# Autodesk Inventor assembly: Robot Assembly
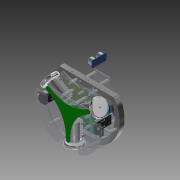
[picture p0: Inventor's stored thumbnail of the model, 180x180]
Saved by Autodesk Inventor 2015 (Build 190159000, 159)
## iProperties
Created: 2016-02-17
Part Number: Robot Assembly
Document SubType Name: Assembly
Designer: 23902
Author: 23902
## Documents named in this file (29)
- C:\Users\23902\git\Work\Design\3D Printing\Version 4\Robot Assembly.iam
- C:\Users\23902\git\Work\Design\3D Printing\Version 4\Motor Mount Plate.ipt
- C:\Users\23902\git\Work\Design\3D Printing\Motor Mount Bracket.ipt
- C:\Users\23902\git\Work\Design\3D Printing\Motor.ipt
- C:\Users\23902\git\Work\Design\3D Printing\Wheel.ipt
- C:\Users\23902\git\Work\Design\3D Printing\Version 4\Middle Plate.ipt
- C:\Users\23902\git\Work\Design\3D Printing\Ball.ipt
- C:\Users\23902\git\Work\Design\3D Printing\Version 4\Standoff 20.ipt
- C:\Users\23902\git\Work\Design\3D Printing\Version 4\Light Sensor Plate.ipt
- C:\Users\23902\git\Work\Design\3D Printing\Version 4\Light Sensor PCB.ipt
- C:\Users\23902\git\Work\Design\3D Printing\Version 4\Standoff 10.ipt
- C:\Users\23902\git\Work\Design\3D Printing\ArduinoMEGA2560.ipt
- C:\Users\23902\git\Work\Design\3D Printing\Version 4\Standoff 30.ipt
- C:\Users\23902\git\Work\Design\3D Printing\Version 4\Veroboard.ipt
- C:\Users\23902\git\Work\Design\3D Printing\Version 4\M3x20 Screw Nylon.ipt
- C:\Users\23902\git\Work\Design\3D Printing\Version 4\M3x10 Screw Nylon.ipt
- C:\Users\23902\git\Work\Design\3D Printing\Version 4\M3x6 Screw Nylon.ipt
- C:\Users\23902\git\Work\Design\3D Printing\Version 4\M3 Nut Nylon.ipt
- C:\Users\23902\git\Work\Design\3D Printing\Version 4\M3x10 Screw Steel.ipt
- C:\Users\23902\git\Work\Design\3D Printing\Version 4\M3 Nut Steel.ipt
- C:\Users\23902\git\Work\Design\3D Printing\Version 4\Battery.ipt
- C:\Users\23902\git\Work\Design\3D Printing\Version 4\Top Plate.ipt
- C:\Users\23902\git\Work\Design\3D Printing\Digit Display.ipt
- C:\Users\23902\git\Work\Design\3D Printing\HC-SR04 Sonar.ipt
- C:\Users\23902\git\Work\Design\3D Printing\Version 4\Sonar Mount.ipt
- C:\Users\23902\git\Work\Design\3D Printing\Version 4\Standoff 40.ipt
- C:\Users\23902\git\Work\Design\3D Printing\Compass.ipt
- C:\Users\23902\git\Work\Design\3D Printing\Version 4\M2x10 Screw Steel.ipt
- C:\Users\23902\git\Work\Design\3D Printing\Version 4\M2 Nut Steel.ipt
## Components (131 placed, 28 different names)
1. Motor Mount Plate:1 — Mate:1, Mate:2, Mate:3, Mate:22, Mate:23, Mate:24, Mate:25, Mate:26, Mate:27, Mate:28, Mate:29, Mate:30, Mate:31, Mate:32, Mate:33, Mate:34, Mate:35, Mate:101, Mate:102, Mate:103, Mate:104, Mate:113, Mate:114, Mate:115, Mate:116, Mate:117, Mate:118, Mate:127, Mate:128, Mate:129, Mate:130, Mate:131, Mate:132, Mate:155, Mate:156, Mate:157, Mate:158, Mate:159, Mate:160, Mate:161, Mate:162, Mate:182, Mate:183, Mate:184, Mate:185, Mate:186, Mate:187, Mate:203, Mate:204, Mate:205, Mate:206, Mate:207, Mate:208, Mate:209, Mate:210, Mate:211, Mate:212, Mate:213, Mate:214, Mate:223, Mate:224, Mate:225, Mate:226, Mate:227, Mate:228, Mate:229, Mate:230, Mate:249, Mate:250, Mate:251, Mate:252, Mate:253, Mate:254, Mate:255, Mate:256, Mate:257, Mate:269, Mate:270, Mate:272, Mate:274, Mate:278, Mate:280, Mate:281, Mate:282, Mate:284, Mate:288, Mate:289, Mate:290, Mate:291, Mate:293, Mate:294, Mate:295, Mate:296, Mate:297, Mate:298, Mate:299, Mate:300, Mate:301, Mate:302, Mate:303
2. Motor Mount Bracket:1 — Mate:1, Mate:11, Mate:14, Mate:15, Mate:24, Mate:25, Mate:275, Mate:276, Mate:286, Mate:287
3. Motor:1 — Mate:10, Mate:16, Mate:17, Mate:21, Flush:3
4. Wheel:1 — Mate:19, Flush:1
5. Motor Mount Bracket:2 — Mate:2, Mate:10, Mate:16, Mate:17, Mate:22, Mate:23, Mate:267, Mate:268, Mate:277, Mate:279
6. Motor:2 — Mate:11, Mate:14, Mate:15, Mate:19, Flush:1
7. Wheel:2 — Mate:20, Flush:2
8. Motor Mount Bracket:3 — Mate:3, Mate:12, Mate:13, Mate:18, Mate:26, Mate:27, Mate:271, Mate:273, Mate:283, Mate:285
9. Motor:3 — Mate:12, Mate:13, Mate:18, Mate:20, Flush:2
10. Wheel:3 — Mate:21, Flush:3
11. Middle Plate:1 — Mate:36, Mate:37, Mate:38, Mate:191, Mate:192, Mate:193, Mate:194, Mate:195, Mate:196, Mate:197, Mate:198, Mate:199, Mate:200, Mate:201, Mate:202, Mate:315, Mate:316, Mate:317, Mate:318, Mate:319, Mate:320, Mate:321, Mate:322, Mate:323, Mate:324, Mate:325, Mate:326, Mate:327, Mate:328, Mate:329, Mate:330
12. Ball:1
13. Standoff 20:1 — Mate:28, Mate:33, Mate:38
14. Standoff 20:2 — Mate:29, Mate:35, Mate:36
15. Standoff 20:3 — Mate:31, Mate:32
16. Standoff 20:4 — Mate:30, Mate:34, Mate:37
17. Light Sensor Plate:1 — Mate:152, Mate:153, Mate:154, Mate:163, Mate:164, Mate:165, Mate:215, Mate:216, Mate:217, Mate:218, Mate:219, Mate:220, Mate:221, Mate:222, Mate:362, Mate:384, Mate:385, Mate:386, Mate:387, Mate:388, Mate:389, Mate:390, Mate:391, Mate:392, Mate:393, Mate:394, Mate:395, Mate:396
18. Light Sensor PCB:1 — Mate:152, Mate:153, Mate:154
19. Standoff 20:5 — Mate:103, Mate:104
20. Standoff 20:6 — Mate:101, Mate:102
21. Standoff 10:1 — Mate:114, Mate:128, Mate:263
22. Standoff 10:2 — Mate:115, Mate:129, Mate:266
23. Standoff 10:3 — Mate:116, Mate:130, Mate:133, Mate:260
24. Standoff 10:4 — Mate:118, Mate:131, Mate:259
25. Standoff 10:5 — Mate:117, Mate:126, Mate:132, Mate:261
26. Standoff 10:6 — Mate:113, Mate:125, Mate:127, Mate:265
27. -  -:1 — Mate:125, Mate:126, Mate:133, Mate:234, Mate:235, Mate:236, Mate:237, Mate:238, Mate:239, Mate:240, Mate:241, Mate:242, Mate:243, Mate:244, Mate:245
28. Standoff 30:1 — Mate:157, Mate:162
29. Standoff 30:2 — Mate:159, Mate:161
30. Standoff 30:3 — Mate:155, Mate:156, Mate:163, Mate:164
31. Standoff 30:4 — Mate:158, Mate:160, Mate:165
32. Standoff 10:7 — Mate:182, Mate:186, Mate:190, Mate:258
33. Standoff 10:8 — Mate:183, Mate:187, Mate:188, Mate:189, Mate:262
34. Standoff 10:9 — Mate:184, Mate:185, Mate:264
35. Veroboard:1 — Mate:188, Mate:189, Mate:190, Mate:231, Mate:232, Mate:233, Mate:246, Mate:247, Mate:248
36. M3x20 Screw Nylon:1 — Mate:192, Mate:201
37. M3x20 Screw Nylon:2 — Mate:193, Mate:202
38. M3x20 Screw Nylon:3 — Mate:194, Mate:199
39. M3x20 Screw Nylon:4 — Mate:195, Mate:198
40. M3x20 Screw Nylon:5 — Mate:196, Mate:197
41. M3x20 Screw Nylon:6 — Mate:191, Mate:200
42. M3x10 Screw Nylon:1 — Mate:208, Mate:209
43. M3x10 Screw Nylon:2 — Mate:207, Mate:210
44. M3x10 Screw Nylon:3 — Mate:206, Mate:211
45. M3x10 Screw Nylon:4 — Mate:205, Mate:212
46. M3x10 Screw Nylon:5 — Mate:204, Mate:213
47. M3x10 Screw Nylon:6 — Mate:203, Mate:214
48. M3x10 Screw Nylon:7 — Mate:215, Mate:219
49. M3x10 Screw Nylon:8 — Mate:216, Mate:220
50. M3x10 Screw Nylon:9 — Mate:224, Mate:225
51. M3x10 Screw Nylon:10 — Mate:218, Mate:222
52. M3x10 Screw Nylon:11 — Mate:217, Mate:221
53. M3x10 Screw Nylon:12 — Mate:228, Mate:229
54. M3x10 Screw Nylon:13 — Mate:227, Mate:230
55. M3x10 Screw Nylon:14 — Mate:223, Mate:226
56. M3x6 Screw Nylon:1 — Mate:231, Mate:246
57. M3x6 Screw Nylon:2 — Mate:235, Mate:240
58. M3x6 Screw Nylon:3 — Mate:236, Mate:242
59. M3x6 Screw Nylon:4 — Mate:237, Mate:245
60. M3x6 Screw Nylon:5 — Mate:239, Mate:244
61. M3x6 Screw Nylon:6 — Mate:238, Mate:241
62. M3x6 Screw Nylon:7 — Mate:232, Mate:247
63. M3x6 Screw Nylon:8 — Mate:234, Mate:243
64. M3x6 Screw Nylon:9 — Mate:233, Mate:248
65. M3 Nut Nylon:1 — Mate:253, Mate:260
66. M3 Nut Nylon:2 — Mate:252, Mate:258
67. M3 Nut Nylon:3 — Mate:254, Mate:262
68. M3 Nut Nylon:4 — Mate:255, Mate:261
69. M3 Nut Nylon:5 — Mate:257, Mate:266
70. M3 Nut Nylon:6 — Mate:256, Mate:264
71. M3 Nut Nylon:7 — Mate:251, Mate:259
72. M3 Nut Nylon:8 — Mate:250, Mate:265
73. M3 Nut Nylon:9 — Mate:249, Mate:263
74. M3x10 Screw Steel:1 — Mate:271, Mate:272, Mate:292
75. M3x10 Screw Steel:2 — Mate:273, Mate:274, Mate:310
76. M3x10 Screw Steel:3 — Mate:268, Mate:269, Mate:307
77. M3x10 Screw Steel:4 — Mate:267, Mate:270, Mate:306
78. M3x10 Screw Steel:5 — Mate:283, Mate:284, Mate:308
79. M3x10 Screw Steel:6 — Mate:279, Mate:280, Mate:304
80. M3x10 Screw Steel:7 — Mate:277, Mate:278, Mate:305
81. M3x10 Screw Steel:8 — Mate:275, Mate:282, Mate:311
82. M3x10 Screw Steel:9 — Mate:287, Mate:288, Mate:314
83. M3x10 Screw Steel:10 — Mate:286, Mate:289, Mate:312
84. M3x10 Screw Steel:11 — Mate:285, Mate:290, Mate:309
85. M3x10 Screw Steel:12 — Mate:276, Mate:281, Mate:313
86. M3 Nut Steel:1 — Mate:295, Mate:314
87. M3 Nut Steel:2 — Mate:291, Mate:292
88. M3 Nut Steel:3 — Mate:294, Mate:312
89. M3 Nut Steel:4 — Mate:296, Mate:311
90. M3 Nut Steel:5 — Mate:298, Mate:310
91. M3 Nut Steel:6 — Mate:297, Mate:304
92. M3 Nut Steel:7 — Mate:300, Mate:305
93. M3 Nut Steel:8 — Mate:299, Mate:308
94. M3 Nut Steel:9 — Mate:301, Mate:306
95. M3 Nut Steel:10 — Mate:302, Mate:309
96. M3 Nut Steel:11 — Mate:293, Mate:313
97. M3 Nut Steel:12 — Mate:303, Mate:307
98. Battery:1
99. Standoff 30:5 — Mate:315, Mate:321
100. Standoff 30:6 — Mate:316, Mate:322, Mate:332
101. Standoff 30:7 — Mate:317, Mate:320, Mate:331, Mate:333
102. Standoff 30:8 — Mate:318, Mate:319
103. M3x20 Screw Nylon:7 — Mate:323, Mate:330
104. M3x20 Screw Nylon:8 — Mate:326, Mate:328
105. M3x20 Screw Nylon:9 — Mate:325, Mate:327
106. M3x20 Screw Nylon:10 — Mate:324, Mate:329
107. Top Plate:1 — Mate:331, Mate:332, Mate:333, Mate:334, Mate:335, Mate:336, Mate:337, Mate:338, Mate:339, Mate:340, Mate:341, Mate:342, Mate:343, Mate:344, Mate:356, Mate:357, Mate:358, Mate:359, Mate:365, Mate:366
108. M3x10 Screw Nylon:15 — Mate:335, Mate:339
109. M3x10 Screw Nylon:16 — Mate:334, Mate:340
110. M3x10 Screw Nylon:17 — Mate:337, Mate:341
111. M3x10 Screw Nylon:18 — Mate:336, Mate:338
112. Digit Display:1 — Mate:342, Mate:343, Mate:344
113. M3x10 Screw Nylon:19 — Mate:357, Mate:359, Mate:368
114. M3x10 Screw Nylon:21 — Mate:356, Mate:358, Mate:367
115. HC-SR04 Sonar:1 — Mate:360, Mate:361, Mate:376, Mate:377, Mate:380, Mate:381
116. Sonar Mount:1 — Mate:360, Mate:361, Mate:362, Mate:384, Mate:385
117. Standoff 40:3 — Mate:366, Mate:367, Mate:371
118. Standoff 40:4 — Mate:365, Mate:368, Mate:369, Mate:370
119. M3x10 Screw Nylon:22 — Mate:373, Mate:374
120. M3x10 Screw Nylon:23 — Mate:372, Mate:375
121. Compass:1 — Mate:369, Mate:370, Mate:371, Mate:372, Mate:373, Mate:374, Mate:375
122. M2x10 Screw Steel:1 — Mate:376, Mate:377, Mate:379
123. M2 Nut Steel:1 — Mate:379
124. M2 Nut Steel:2 — Mate:383
125. M2x10 Screw Steel:2 — Mate:380, Mate:381, Mate:383
126. HC-SR04 Sonar:2
127. Sonar Mount:2 — Mate:386, Mate:387, Mate:388
128. M3x10 Screw Nylon:24 — Mate:394, Mate:396
129. M3x10 Screw Nylon:25 — Mate:393, Mate:395
130. M3x10 Screw Nylon:26 — Mate:389, Mate:390
131. M3x10 Screw Nylon:27 — Mate:391, Mate:392
## Relationships (268: Mate 265, Flush 3)
- Mate:1: Motor Mount Plate:1 ↔ Motor Mount Bracket:1
- Mate:2: Motor Mount Plate:1 ↔ Motor Mount Bracket:2
- Mate:3: Motor Mount Plate:1 ↔ Motor Mount Bracket:3
- Mate:10: Motor:1 ↔ Motor Mount Bracket:2
- Mate:11: Motor Mount Bracket:1 ↔ Motor:2
- Mate:12: Motor Mount Bracket:3 ↔ Motor:3
- Mate:13: Motor Mount Bracket:3 ↔ Motor:3
- Mate:14: Motor Mount Bracket:1 ↔ Motor:2
- Mate:15: Motor Mount Bracket:1 ↔ Motor:2
- Mate:16: Motor:1 ↔ Motor Mount Bracket:2
- Mate:17: Motor:1 ↔ Motor Mount Bracket:2
- Mate:18: Motor Mount Bracket:3 ↔ Motor:3
- Mate:19: Wheel:1 ↔ Motor:2
- Flush:1: Wheel:1 ↔ Motor:2
- Mate:20: Wheel:2 ↔ Motor:3
- Flush:2: Wheel:2 ↔ Motor:3
- Mate:21: Motor:1 ↔ Wheel:3
- Flush:3: Motor:1 ↔ Wheel:3
- Mate:22: Motor Mount Plate:1 ↔ Motor Mount Bracket:2
- Mate:23: Motor Mount Plate:1 ↔ Motor Mount Bracket:2
- Mate:24: Motor Mount Plate:1 ↔ Motor Mount Bracket:1
- Mate:25: Motor Mount Plate:1 ↔ Motor Mount Bracket:1
- Mate:26: Motor Mount Plate:1 ↔ Motor Mount Bracket:3
- Mate:27: Motor Mount Plate:1 ↔ Motor Mount Bracket:3
- Mate:28: Motor Mount Plate:1 ↔ Standoff 20:1
- Mate:29: Motor Mount Plate:1 ↔ Standoff 20:2
- Mate:30: Motor Mount Plate:1 ↔ Standoff 20:4
- Mate:31: Motor Mount Plate:1 ↔ Standoff 20:3
- Mate:32: Motor Mount Plate:1 ↔ Standoff 20:3
- Mate:33: Motor Mount Plate:1 ↔ Standoff 20:1
- Mate:34: Motor Mount Plate:1 ↔ Standoff 20:4
- Mate:35: Motor Mount Plate:1 ↔ Standoff 20:2
- Mate:36: Middle Plate:1 ↔ Standoff 20:2
- Mate:37: Middle Plate:1 ↔ Standoff 20:4
- Mate:38: Middle Plate:1 ↔ Standoff 20:1
- Mate:101: Motor Mount Plate:1 ↔ Standoff 20:6
- Mate:102: Motor Mount Plate:1 ↔ Standoff 20:6
- Mate:103: Motor Mount Plate:1 ↔ Standoff 20:5
- Mate:104: Motor Mount Plate:1 ↔ Standoff 20:5
- Mate:113: Motor Mount Plate:1 ↔ Standoff 10:6
- Mate:114: Motor Mount Plate:1 ↔ Standoff 10:1
- Mate:115: Motor Mount Plate:1 ↔ Standoff 10:2
- Mate:116: Motor Mount Plate:1 ↔ Standoff 10:3
- Mate:117: Motor Mount Plate:1 ↔ Standoff 10:5
- Mate:118: Motor Mount Plate:1 ↔ Standoff 10:4
- Mate:125: Standoff 10:6 ↔ -  -:1
- Mate:126: Standoff 10:5 ↔ -  -:1
- Mate:127: Motor Mount Plate:1 ↔ Standoff 10:6
- Mate:128: Motor Mount Plate:1 ↔ Standoff 10:1
- Mate:129: Motor Mount Plate:1 ↔ Standoff 10:2
- Mate:130: Motor Mount Plate:1 ↔ Standoff 10:3
- Mate:131: Motor Mount Plate:1 ↔ Standoff 10:4
- Mate:132: Motor Mount Plate:1 ↔ Standoff 10:5
- Mate:133: Standoff 10:3 ↔ -  -:1
- Mate:152: Light Sensor Plate:1 ↔ Light Sensor PCB:1
- Mate:153: Light Sensor Plate:1 ↔ Light Sensor PCB:1
- Mate:154: Light Sensor Plate:1 ↔ Light Sensor PCB:1
- Mate:155: Motor Mount Plate:1 ↔ Standoff 30:3
- Mate:156: Motor Mount Plate:1 ↔ Standoff 30:3
- Mate:157: Motor Mount Plate:1 ↔ Standoff 30:1
- Mate:158: Motor Mount Plate:1 ↔ Standoff 30:4
- Mate:159: Motor Mount Plate:1 ↔ Standoff 30:2
- Mate:160: Motor Mount Plate:1 ↔ Standoff 30:4
- Mate:161: Motor Mount Plate:1 ↔ Standoff 30:2
- Mate:162: Motor Mount Plate:1 ↔ Standoff 30:1
- Mate:163: Light Sensor Plate:1 ↔ Standoff 30:3
- Mate:164: Light Sensor Plate:1 ↔ Standoff 30:3
- Mate:165: Light Sensor Plate:1 ↔ Standoff 30:4
- Mate:182: Motor Mount Plate:1 ↔ Standoff 10:7
- Mate:183: Motor Mount Plate:1 ↔ Standoff 10:8
- Mate:184: Motor Mount Plate:1 ↔ Standoff 10:9
- Mate:185: Motor Mount Plate:1 ↔ Standoff 10:9
- Mate:186: Motor Mount Plate:1 ↔ Standoff 10:7
- Mate:187: Motor Mount Plate:1 ↔ Standoff 10:8
- Mate:188: Standoff 10:8 ↔ Veroboard:1
- Mate:189: Standoff 10:8 ↔ Veroboard:1
- Mate:190: Standoff 10:7 ↔ Veroboard:1
- Mate:191: Middle Plate:1 ↔ M3x20 Screw Nylon:6
- Mate:192: Middle Plate:1 ↔ M3x20 Screw Nylon:1
- Mate:193: Middle Plate:1 ↔ M3x20 Screw Nylon:2
- Mate:194: Middle Plate:1 ↔ M3x20 Screw Nylon:3
- Mate:195: Middle Plate:1 ↔ M3x20 Screw Nylon:4
- Mate:196: Middle Plate:1 ↔ M3x20 Screw Nylon:5
- Mate:197: Middle Plate:1 ↔ M3x20 Screw Nylon:5
- Mate:198: Middle Plate:1 ↔ M3x20 Screw Nylon:4
- Mate:199: Middle Plate:1 ↔ M3x20 Screw Nylon:3
- Mate:200: Middle Plate:1 ↔ M3x20 Screw Nylon:6
- Mate:201: Middle Plate:1 ↔ M3x20 Screw Nylon:1
- Mate:202: Middle Plate:1 ↔ M3x20 Screw Nylon:2
- Mate:203: Motor Mount Plate:1 ↔ M3x10 Screw Nylon:6
- Mate:204: Motor Mount Plate:1 ↔ M3x10 Screw Nylon:5
- Mate:205: Motor Mount Plate:1 ↔ M3x10 Screw Nylon:4
- Mate:206: Motor Mount Plate:1 ↔ M3x10 Screw Nylon:3
- Mate:207: Motor Mount Plate:1 ↔ M3x10 Screw Nylon:2
- Mate:208: Motor Mount Plate:1 ↔ M3x10 Screw Nylon:1
- Mate:209: Motor Mount Plate:1 ↔ M3x10 Screw Nylon:1
- Mate:210: Motor Mount Plate:1 ↔ M3x10 Screw Nylon:2
- Mate:211: Motor Mount Plate:1 ↔ M3x10 Screw Nylon:3
- Mate:212: Motor Mount Plate:1 ↔ M3x10 Screw Nylon:4
- Mate:213: Motor Mount Plate:1 ↔ M3x10 Screw Nylon:5
- Mate:214: Motor Mount Plate:1 ↔ M3x10 Screw Nylon:6
- Mate:215: Light Sensor Plate:1 ↔ M3x10 Screw Nylon:7
- Mate:216: Light Sensor Plate:1 ↔ M3x10 Screw Nylon:8
- Mate:217: Light Sensor Plate:1 ↔ M3x10 Screw Nylon:11
- Mate:218: Light Sensor Plate:1 ↔ M3x10 Screw Nylon:10
- Mate:219: Light Sensor Plate:1 ↔ M3x10 Screw Nylon:7
- Mate:220: Light Sensor Plate:1 ↔ M3x10 Screw Nylon:8
- Mate:221: Light Sensor Plate:1 ↔ M3x10 Screw Nylon:11
- Mate:222: Light Sensor Plate:1 ↔ M3x10 Screw Nylon:10
- Mate:223: Motor Mount Plate:1 ↔ M3x10 Screw Nylon:14
- Mate:224: Motor Mount Plate:1 ↔ M3x10 Screw Nylon:9
- Mate:225: Motor Mount Plate:1 ↔ M3x10 Screw Nylon:9
- Mate:226: Motor Mount Plate:1 ↔ M3x10 Screw Nylon:14
- Mate:227: Motor Mount Plate:1 ↔ M3x10 Screw Nylon:13
- Mate:228: Motor Mount Plate:1 ↔ M3x10 Screw Nylon:12
- Mate:229: Motor Mount Plate:1 ↔ M3x10 Screw Nylon:12
- Mate:230: Motor Mount Plate:1 ↔ M3x10 Screw Nylon:13
- Mate:231: Veroboard:1 ↔ M3x6 Screw Nylon:1
- Mate:232: Veroboard:1 ↔ M3x6 Screw Nylon:7
- Mate:233: Veroboard:1 ↔ M3x6 Screw Nylon:9
- Mate:234: -  -:1 ↔ M3x6 Screw Nylon:8
- Mate:235: -  -:1 ↔ M3x6 Screw Nylon:2
- Mate:236: -  -:1 ↔ M3x6 Screw Nylon:3
- Mate:237: -  -:1 ↔ M3x6 Screw Nylon:4
- Mate:238: -  -:1 ↔ M3x6 Screw Nylon:6
- Mate:239: -  -:1 ↔ M3x6 Screw Nylon:5
- Mate:240: -  -:1 ↔ M3x6 Screw Nylon:2
- Mate:241: -  -:1 ↔ M3x6 Screw Nylon:6
- Mate:242: -  -:1 ↔ M3x6 Screw Nylon:3
- Mate:243: -  -:1 ↔ M3x6 Screw Nylon:8
- Mate:244: -  -:1 ↔ M3x6 Screw Nylon:5
- Mate:245: -  -:1 ↔ M3x6 Screw Nylon:4
- Mate:246: Veroboard:1 ↔ M3x6 Screw Nylon:1
- Mate:247: Veroboard:1 ↔ M3x6 Screw Nylon:7
- Mate:248: Veroboard:1 ↔ M3x6 Screw Nylon:9
- Mate:249: Motor Mount Plate:1 ↔ M3 Nut Nylon:9
- Mate:250: Motor Mount Plate:1 ↔ M3 Nut Nylon:8
- Mate:251: Motor Mount Plate:1 ↔ M3 Nut Nylon:7
- Mate:252: Motor Mount Plate:1 ↔ M3 Nut Nylon:2
- Mate:253: Motor Mount Plate:1 ↔ M3 Nut Nylon:1
- Mate:254: Motor Mount Plate:1 ↔ M3 Nut Nylon:3
- Mate:255: Motor Mount Plate:1 ↔ M3 Nut Nylon:4
- Mate:256: Motor Mount Plate:1 ↔ M3 Nut Nylon:6
- Mate:257: Motor Mount Plate:1 ↔ M3 Nut Nylon:5
- Mate:258: Standoff 10:7 ↔ M3 Nut Nylon:2
- Mate:259: Standoff 10:4 ↔ M3 Nut Nylon:7
- Mate:260: Standoff 10:3 ↔ M3 Nut Nylon:1
- Mate:261: Standoff 10:5 ↔ M3 Nut Nylon:4
- Mate:262: Standoff 10:8 ↔ M3 Nut Nylon:3
- Mate:263: Standoff 10:1 ↔ M3 Nut Nylon:9
- Mate:264: Standoff 10:9 ↔ M3 Nut Nylon:6
- Mate:265: Standoff 10:6 ↔ M3 Nut Nylon:8
- Mate:266: Standoff 10:2 ↔ M3 Nut Nylon:5
- Mate:267: Motor Mount Bracket:2 ↔ M3x10 Screw Steel:4
- Mate:268: Motor Mount Bracket:2 ↔ M3x10 Screw Steel:3
- Mate:269: Motor Mount Plate:1 ↔ M3x10 Screw Steel:3
- Mate:270: Motor Mount Plate:1 ↔ M3x10 Screw Steel:4
- Mate:271: Motor Mount Bracket:3 ↔ M3x10 Screw Steel:1
- Mate:272: Motor Mount Plate:1 ↔ M3x10 Screw Steel:1
- Mate:273: Motor Mount Bracket:3 ↔ M3x10 Screw Steel:2
- Mate:274: Motor Mount Plate:1 ↔ M3x10 Screw Steel:2
- Mate:275: Motor Mount Bracket:1 ↔ M3x10 Screw Steel:8
- Mate:276: Motor Mount Bracket:1 ↔ M3x10 Screw Steel:12
- Mate:277: Motor Mount Bracket:2 ↔ M3x10 Screw Steel:7
- Mate:278: Motor Mount Plate:1 ↔ M3x10 Screw Steel:7
- Mate:279: Motor Mount Bracket:2 ↔ M3x10 Screw Steel:6
- Mate:280: Motor Mount Plate:1 ↔ M3x10 Screw Steel:6
- Mate:281: Motor Mount Plate:1 ↔ M3x10 Screw Steel:12
- Mate:282: Motor Mount Plate:1 ↔ M3x10 Screw Steel:8
- Mate:283: Motor Mount Bracket:3 ↔ M3x10 Screw Steel:5
- Mate:284: Motor Mount Plate:1 ↔ M3x10 Screw Steel:5
- Mate:285: Motor Mount Bracket:3 ↔ M3x10 Screw Steel:11
- Mate:286: Motor Mount Bracket:1 ↔ M3x10 Screw Steel:10
- Mate:287: Motor Mount Bracket:1 ↔ M3x10 Screw Steel:9
- Mate:288: Motor Mount Plate:1 ↔ M3x10 Screw Steel:9
- Mate:289: Motor Mount Plate:1 ↔ M3x10 Screw Steel:10
- Mate:290: Motor Mount Plate:1 ↔ M3x10 Screw Steel:11
- Mate:291: Motor Mount Plate:1 ↔ M3 Nut Steel:2
- Mate:292: M3x10 Screw Steel:1 ↔ M3 Nut Steel:2
- Mate:293: Motor Mount Plate:1 ↔ M3 Nut Steel:11
- Mate:294: Motor Mount Plate:1 ↔ M3 Nut Steel:3
- Mate:295: Motor Mount Plate:1 ↔ M3 Nut Steel:1
- Mate:296: Motor Mount Plate:1 ↔ M3 Nut Steel:4
- Mate:297: Motor Mount Plate:1 ↔ M3 Nut Steel:6
- Mate:298: Motor Mount Plate:1 ↔ M3 Nut Steel:5
- Mate:299: Motor Mount Plate:1 ↔ M3 Nut Steel:8
- Mate:300: Motor Mount Plate:1 ↔ M3 Nut Steel:7
- Mate:301: Motor Mount Plate:1 ↔ M3 Nut Steel:9
- Mate:302: Motor Mount Plate:1 ↔ M3 Nut Steel:10
- Mate:303: Motor Mount Plate:1 ↔ M3 Nut Steel:12
- Mate:304: M3x10 Screw Steel:6 ↔ M3 Nut Steel:6
- Mate:305: M3x10 Screw Steel:7 ↔ M3 Nut Steel:7
- Mate:306: M3x10 Screw Steel:4 ↔ M3 Nut Steel:9
- Mate:307: M3x10 Screw Steel:3 ↔ M3 Nut Steel:12
- Mate:308: M3x10 Screw Steel:5 ↔ M3 Nut Steel:8
- Mate:309: M3x10 Screw Steel:11 ↔ M3 Nut Steel:10
- Mate:310: M3x10 Screw Steel:2 ↔ M3 Nut Steel:5
- Mate:311: M3x10 Screw Steel:8 ↔ M3 Nut Steel:4
- Mate:312: M3x10 Screw Steel:10 ↔ M3 Nut Steel:3
- Mate:313: M3x10 Screw Steel:12 ↔ M3 Nut Steel:11
- Mate:314: M3x10 Screw Steel:9 ↔ M3 Nut Steel:1
- Mate:315: Middle Plate:1 ↔ Standoff 30:5
- Mate:316: Middle Plate:1 ↔ Standoff 30:6
- Mate:317: Middle Plate:1 ↔ Standoff 30:7
- Mate:318: Middle Plate:1 ↔ Standoff 30:8
- Mate:319: Middle Plate:1 ↔ Standoff 30:8
- Mate:320: Middle Plate:1 ↔ Standoff 30:7
- Mate:321: Middle Plate:1 ↔ Standoff 30:5
- Mate:322: Middle Plate:1 ↔ Standoff 30:6
- Mate:323: Middle Plate:1 ↔ M3x20 Screw Nylon:7
- Mate:324: Middle Plate:1 ↔ M3x20 Screw Nylon:10
- Mate:325: Middle Plate:1 ↔ M3x20 Screw Nylon:9
- Mate:326: Middle Plate:1 ↔ M3x20 Screw Nylon:8
- Mate:327: Middle Plate:1 ↔ M3x20 Screw Nylon:9
- Mate:328: Middle Plate:1 ↔ M3x20 Screw Nylon:8
- Mate:329: Middle Plate:1 ↔ M3x20 Screw Nylon:10
- Mate:330: Middle Plate:1 ↔ M3x20 Screw Nylon:7
- Mate:331: Standoff 30:7 ↔ Top Plate:1
- Mate:332: Standoff 30:6 ↔ Top Plate:1
- Mate:333: Standoff 30:7 ↔ Top Plate:1
- Mate:334: Top Plate:1 ↔ M3x10 Screw Nylon:16
- Mate:335: Top Plate:1 ↔ M3x10 Screw Nylon:15
- Mate:336: Top Plate:1 ↔ M3x10 Screw Nylon:18
- Mate:337: Top Plate:1 ↔ M3x10 Screw Nylon:17
- Mate:338: Top Plate:1 ↔ M3x10 Screw Nylon:18
- Mate:339: Top Plate:1 ↔ M3x10 Screw Nylon:15
- Mate:340: Top Plate:1 ↔ M3x10 Screw Nylon:16
- Mate:341: Top Plate:1 ↔ M3x10 Screw Nylon:17
- Mate:342 (2 mm): Top Plate:1 ↔ Digit Display:1
- Mate:343 (0.5 mm): Top Plate:1 ↔ Digit Display:1
- Mate:344 (2 mm): Top Plate:1 ↔ Digit Display:1
- Mate:356: Top Plate:1 ↔ M3x10 Screw Nylon:21
- Mate:357: Top Plate:1 ↔ M3x10 Screw Nylon:19
- Mate:358: Top Plate:1 ↔ M3x10 Screw Nylon:21
- Mate:359: Top Plate:1 ↔ M3x10 Screw Nylon:19
- Mate:360 (1 mm): HC-SR04 Sonar:1 ↔ Sonar Mount:1
- Mate:361: HC-SR04 Sonar:1 ↔ Sonar Mount:1
- Mate:362: Light Sensor Plate:1 ↔ Sonar Mount:1
- Mate:365: Top Plate:1 ↔ Standoff 40:4
- Mate:366: Top Plate:1 ↔ Standoff 40:3
- Mate:367: M3x10 Screw Nylon:21 ↔ Standoff 40:3
- Mate:368: M3x10 Screw Nylon:19 ↔ Standoff 40:4
- Mate:369: Standoff 40:4 ↔ Compass:1
- Mate:370: Standoff 40:4 ↔ Compass:1
- Mate:371: Standoff 40:3 ↔ Compass:1
- Mate:372: M3x10 Screw Nylon:23 ↔ Compass:1
- Mate:373: M3x10 Screw Nylon:22 ↔ Compass:1
- Mate:374: M3x10 Screw Nylon:22 ↔ Compass:1
- Mate:375: M3x10 Screw Nylon:23 ↔ Compass:1
- Mate:376: HC-SR04 Sonar:1 ↔ M2x10 Screw Steel:1
- Mate:377: HC-SR04 Sonar:1 ↔ M2x10 Screw Steel:1
- Mate:379: M2x10 Screw Steel:1 ↔ M2 Nut Steel:1
- Mate:380: HC-SR04 Sonar:1 ↔ M2x10 Screw Steel:2
- Mate:381: HC-SR04 Sonar:1 ↔ M2x10 Screw Steel:2
- Mate:383: M2 Nut Steel:2 ↔ M2x10 Screw Steel:2
- Mate:384: Light Sensor Plate:1 ↔ Sonar Mount:1
- Mate:385: Light Sensor Plate:1 ↔ Sonar Mount:1
- Mate:386: Light Sensor Plate:1 ↔ Sonar Mount:2
- Mate:387: Light Sensor Plate:1 ↔ Sonar Mount:2
- Mate:388: Light Sensor Plate:1 ↔ Sonar Mount:2
- Mate:389: Light Sensor Plate:1 ↔ M3x10 Screw Nylon:26
- Mate:390: Light Sensor Plate:1 ↔ M3x10 Screw Nylon:26
- Mate:391: Light Sensor Plate:1 ↔ M3x10 Screw Nylon:27
- Mate:392: Light Sensor Plate:1 ↔ M3x10 Screw Nylon:27
- Mate:393: Light Sensor Plate:1 ↔ M3x10 Screw Nylon:25
- Mate:394: Light Sensor Plate:1 ↔ M3x10 Screw Nylon:24
- Mate:395: Light Sensor Plate:1 ↔ M3x10 Screw Nylon:25
- Mate:396: Light Sensor Plate:1 ↔ M3x10 Screw Nylon:24
